# Autodesk Inventor assembly: door_hinge
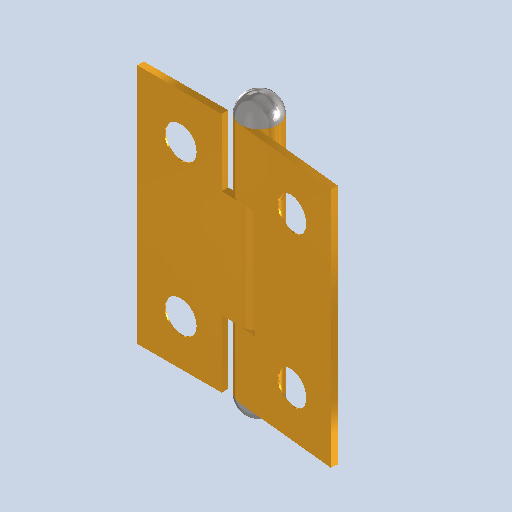
[picture p0: Inventor's stored thumbnail of the model, 512x512]
Saved by Autodesk Inventor 2023.2 (Build 272271030, 271C)
## iProperties
Created: 2022-08-13
Part Number: door_hinge
Document SubType Name: Assembly
Designer: User
Author: User
## Documents named in this file (4)
- D:\!project\fox_n_crow_construction\crow\face\door_hinge.iam
- D:\!project\fox_n_crow_construction\crow\face\hinge_component1.ipt
- D:\!project\fox_n_crow_construction\crow\face\hinge_axis.ipt
- D:\!project\fox_n_crow_construction\crow\face\hinge_component2.ipt
## Components (3 placed, 3 different names)
1. hinge_component1:1 — Совмещение:2, Заподлицо:1, Заподлицо:2
2. hinge_axis:1 — Совмещение:1, Совмещение:2, Заподлицо:2
3. hinge_component2:1 — Совмещение:1, Заподлицо:1
## Relationships (4: Mate 2, Flush 2)
- Совмещение:1 [Mate]: hinge_axis:1 ↔ hinge_component2:1
- Совмещение:2 [Mate]: hinge_component1:1 ↔ hinge_axis:1
- Заподлицо:1 [Flush]: hinge_component1:1 ↔ hinge_component2:1
- Заподлицо:2 [Flush]: hinge_component1:1 ↔ hinge_axis:1
